# Autodesk Inventor assembly: Center Tower 4.4r
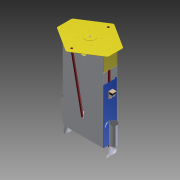
[picture p0: Inventor's stored thumbnail of the model, 180x180]
Saved by Autodesk Inventor 2015 (Build 190159000, 159)
## iProperties
Created: 2015-04-21
Part Number: Center Tower 4.4r
Document SubType Name: Assembly
Designer: David Tenney
Author: David Tenney
## Documents named in this file (26)
- C:\Users\David Tenney\Documents\GitHub\CAD\Field\Imported Components\Full_Field_V5.3_Full_Detail\Center Tower 4.4r.iam
- C:\Users\David Tenney\Documents\GitHub\CAD\Field\Imported Components\Full_Field_V5.3_Full_Detail\Upper Cross Brace reverse.ipt
- C:\Users\David Tenney\Documents\GitHub\CAD\Field\Imported Components\Full_Field_V5.3_Full_Detail\Side Panel Upper Reverse.ipt
- C:\Users\David Tenney\Documents\GitHub\CAD\Field\Imported Components\Full_Field_V5.3_Full_Detail\Splitter Ramp v2.ipt
- C:\Users\David Tenney\Documents\GitHub\CAD\Field\Imported Components\Full_Field_V5.3_Full_Detail\Front panel v2.ipt
- C:\Users\David Tenney\Documents\GitHub\CAD\Field\Imported Components\Full_Field_V5.3_Full_Detail\Ball Tray v4.ipt
- C:\Users\David Tenney\Documents\GitHub\CAD\Field\Imported Components\Full_Field_V5.3_Full_Detail\Floor plate.ipt
- C:\Users\David Tenney\Documents\GitHub\CAD\Field\Imported Components\Full_Field_V5.3_Full_Detail\Bracket 90 - Bolt Bottom.ipt
- C:\Users\David Tenney\Documents\GitHub\CAD\Field\Imported Components\Full_Field_V5.3_Full_Detail\Pipe Diverter.ipt
- C:\Users\David Tenney\Documents\GitHub\CAD\Field\Imported Components\Full_Field_V5.3_Full_Detail\Pipe v4.ipt
- C:\Users\David Tenney\Documents\GitHub\CAD\Field\Imported Components\Full_Field_V5.3_Full_Detail\ASM_NEW_IRBEACON_ASM.iam
- C:\Users\David Tenney\Documents\GitHub\CAD\Field\Imported Components\Full_Field_V5.3_Full_Detail\0_125 rivet.ipt
- C:\Users\David Tenney\Documents\GitHub\CAD\Field\Imported Components\Full_Field_V5.3_Full_Detail\10-32 x 0_375 BHCS.ipt
- C:\Users\David Tenney\Documents\GitHub\CAD\Field\Imported Components\Full_Field_V5.3_Full_Detail\10-32 Nylock Jam Nut_90633A411.ipt
- C:\Users\David Tenney\Documents\GitHub\CAD\Field\Imported Components\Full_Field_V5.3_Full_Detail\Bracket 90.ipt
- C:\Users\David Tenney\Documents\GitHub\CAD\Field\Imported Components\Full_Field_V5.3_Full_Detail\socket head cap screw_ai_HX-SHCS 0.19-32x1.375x1-C.ipt
- C:\Users\David Tenney\Documents\GitHub\CAD\Field\Imported Components\Full_Field_V5.3_Full_Detail\10-32x1250_shcs.ipt
- C:\Users\David Tenney\Documents\GitHub\CAD\Field\Imported Components\Full_Field_V5.3_Full_Detail\Upper goal tube.iam
- C:\Users\David Tenney\Documents\GitHub\CAD\Field\Imported Components\Full_Field_V5.3_Full_Detail\elevator screw 1.25in.ipt
- C:\Users\David Tenney\Documents\GitHub\CAD\Field\Imported Components\Full_Field_V5.3_Full_Detail\Center Pivot Plate.ipt
- C:\Users\David Tenney\Documents\GitHub\CAD\Field\Imported Components\Full_Field_V5.3_Full_Detail\14-20 NyLock thin - Mcm 90566A029_90566A029.ipt
- C:\Users\David Tenney\Documents\GitHub\CAD\Field\Imported Components\Full_Field_V5.3_Full_Detail\10-32x1000_shcs_HX-SHCS 0.19-32x1.375x1-C.ipt
- C:\Users\David Tenney\Documents\GitHub\CAD\Field\Imported Components\Full_Field_V5.3_Full_Detail\IR Beacon Hanger.ipt
- C:\Users\David Tenney\Documents\GitHub\CAD\Field\Side Panel Upper Reverse Red.ipt
- C:\Users\David Tenney\Documents\GitHub\CAD\Field\Pipe v4 blue.ipt
- C:\Users\David Tenney\Documents\GitHub\CAD\Field\Imported Components\Full_Field_V5.3_Full_Detail\Front panel v2 Clear.ipt
## Components (96 placed, 96 different names)
1. Upper Cross Brace reverse_172
2. Side Panel Upper Reverse_173 — Symmetry:2
3. Side Panel Upper Reverse_174 — Symmetry:2
4. Splitter Ramp v2_175
5. Front panel v2_176 — Symmetry:1
6. Ball Tray v4_177
7. Ball Tray v4_178
8. Floor plate_179 — Flush:1
9. Bracket 90 - Bolt Bottom_180
10. Bracket 90 - Bolt Bottom_181
11. Bracket 90 - Bolt Bottom_182
12. Bracket 90 - Bolt Bottom_183
13. Front panel v2_184 — Symmetry:1
14. Pipe Diverter_185
15. Pipe Diverter_186
16. Pipe v4_187
17. Pipe v4_188
18. ASM_NEW_IRBEACON_ASM_189 [sub-assembly]
19. ASM_NEW_IRBEACON_ASM_190 [sub-assembly]
20. Bracket 90 - Bolt Bottom_191
21. Bracket 90 - Bolt Bottom_192
22. 0_125 rivet_193
23. 0_125 rivet_194
24. 0_125 rivet_195
25. 0_125 rivet_196
26. 0_125 rivet_197
27. 0_125 rivet_198
28. 0_125 rivet_199
29. 0_125 rivet_200
30. 0_125 rivet_201
31. 0_125 rivet_202
32. 10-32 x 0_375 BHCS_203
33. 10-32 Nylock Jam Nut_90633A411_204
34. 10-32 Nylock Jam Nut_90633A411_205
35. 10-32 x 0_375 BHCS_206
36. Bracket 90_207
37. Bracket 90_208
38. 0_125 rivet_209
39. 0_125 rivet_210
40. 0_125 rivet_211
41. 0_125 rivet_212
42. 0_125 rivet_213
43. 0_125 rivet_214
44. 0_125 rivet_215
45. 0_125 rivet_216
46. 0_125 rivet_217
47. 0_125 rivet_218
48. 0_125 rivet_219
49. 0_125 rivet_220
50. 0_125 rivet_221
51. 0_125 rivet_222
52. 0_125 rivet_223
53. 0_125 rivet_224
54. 0_125 rivet_225
55. 0_125 rivet_226
56. 0_125 rivet_227
57. 0_125 rivet_228
58. 0_125 rivet_229
59. 0_125 rivet_230
60. 0_125 rivet_231
61. 0_125 rivet_232
62. 0_125 rivet_233
63. 0_125 rivet_234
64. socket head cap screw_ai_HX-SHCS 0.19-32x1.375x1-C_235
65. socket head cap screw_ai_HX-SHCS 0.19-32x1.375x1-C_236
66. 10-32x1250_shcs_237
67. 10-32x1250_shcs_238
68. 10-32 Nylock Jam Nut_90633A411_239
69. 10-32 Nylock Jam Nut_90633A411_240
70. 10-32 Nylock Jam Nut_90633A411_241
71. 10-32 Nylock Jam Nut_90633A411_242
72. Upper goal tube_243 [sub-assembly]
73. Upper goal tube_244 [sub-assembly]
74. 0_125 rivet_245
75. 0_125 rivet_246
76. 0_125 rivet_247
77. 0_125 rivet_248
78. 10-32 x 0_375 BHCS_249
79. 10-32 x 0_375 BHCS_250
80. 10-32 x 0_375 BHCS_251
81. 10-32 x 0_375 BHCS_252
82. 10-32 Nylock Jam Nut_90633A411_253
83. 10-32 Nylock Jam Nut_90633A411_254
84. 10-32 Nylock Jam Nut_90633A411_255
85. 10-32 Nylock Jam Nut_90633A411_256
86. elevator screw 1.25in_257
87. Center Pivot Plate_258
88. 14-20 NyLock thin - Mcm 90566A029_90566A029_259
89. 10-32 Nylock Jam Nut_90633A411_260
90. 10-32 Nylock Jam Nut_90633A411_261
91. 10-32 Nylock Jam Nut_90633A411_262
92. 10-32 Nylock Jam Nut_90633A411_263
93. 10-32x1000_shcs_HX-SHCS 0.19-32x1.375x1-C_264
94. 10-32x1000_shcs_HX-SHCS 0.19-32x1.375x1-C_265
95. IR Beacon Hanger_266
96. IR Beacon Hanger_267
## Relationships (5: Symmetry 2, Mate 2, Flush 1)
- Symmetry:1: Front panel v2_176 ↔ Front panel v2_184
- Symmetry:2: Side Panel Upper Reverse_173 ↔ Side Panel Upper Reverse_174
- Flush:1 (-301.625 mm): Floor plate_179
- Mate:1
- Mate:2
